# Autodesk Inventor assembly: WheelAssembly3.0
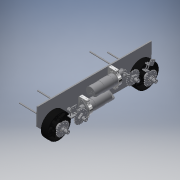
[picture p0: Inventor's stored thumbnail of the model, 180x180]
Saved by Autodesk Inventor 2017 (Build 210142000, 142)
## iProperties
Created: 2017-07-22
Part Number: WheelAssembly3.0
Document SubType Name: Assembly
Designer: User
Author: User
## Documents named in this file (17)
- C:\Robotics\CAD\2018-19_CAD\InvertedDriveTrain.iam
- C:\Robotics\CAD\COTSParts\Motors\Andymark 2964  NeveRest 40 Motor.ipt
- C:\Robotics\CAD\COTSParts\Tetrix\tetrix-motor-mounts-1.snapshot.1\Tetrex 2pc motor mount.ipt
- C:\Robotics\CAD\COTSParts\Actobotics\615 parts\615398.25inBoreBeveledGears.ipt
- C:\Robotics\CAD\2016-17_CAD\Custom COTS\4inax.ipt
- C:\Robotics\CAD\COTSParts\Actobotics\615 parts\615106Sprocket.5inBore.25inPitch24Teeth.ipt
- C:\Robotics\CAD\COTSParts\Actobotics\545 parts\545556SetScrewHub.77inPattern.ipt
- C:\Robotics\CAD\COTSParts\Wheels\4in Wheel Intergreated Hub 8mm Rev2.ipt
- C:\Robotics\CAD\COTSParts\Actobotics\Thrust Bearings\6655K13.ipt
- C:\Robotics\CAD\2018-19_CAD\InvertedDrivePlateOutside.ipt
- C:\Robotics\CAD\2018-19_CAD\InvertedDrivePlateInside.ipt
- C:\Robotics\CAD\2018-19_CAD\Offseason\WheelandSprocketComboHub2.ipt
- C:\Robotics\CAD\COTSParts\Actobotics\535 parts\535198Bearing.25ID.5OD.ipt
- C:\Robotics\CAD\2018-19_CAD\Offseason\Tensioner3.iam
- C:\Robotics\CAD\2018-19_CAD\Offseason\MotorFixedPositionMountInvertedDrive.ipt
- C:\Robotics\CAD\COTSParts\Actobotics\Collar.ipt
- C:\Robotics\CAD\COTSParts\Fasteners\6-32 SHCS x500.ipt
## Components (56 placed, 16 different names)
1. Andymark 2964  NeveRest 40 Motor:1 — Insert:3, Insert:6
2. Andymark 2964  NeveRest 40 Motor:2 — Insert:4, Insert:5
3. Tetrex 2pc motor mount:1 — Insert:3, Insert:79, Angle:8, Insert:84
4. Tetrex 2pc motor mount:2 — Insert:4, Insert:80, Angle:9, Insert:85
5. 615398.25inBoreBeveledGears:1 — Insert:5, Insert:44
6. 615398.25inBoreBeveledGears:2 — Insert:6, Insert:47
7. 615398.25inBoreBeveledGears:3 — Insert:77
8. 615398.25inBoreBeveledGears:4 — Insert:78
9. 4inax:1 — Insert:60, Mate:30
10. 4inax:2 — Insert:61
11. 615106Sprocket.5inBore.25inPitch24Teeth:2 — Insert:102, Insert:103, Insert:104
12. 4inax:3 — Insert:58, Mate:29
13. 4inax:4 — Insert:59
14. 545556SetScrewHub.77inPattern:4 — Insert:54
15. 4in Wheel Intergreated Hub 8mm Rev2:1 — Insert:65
16. 4in Wheel Intergreated Hub 8mm Rev2:2 — Insert:68
17. 545556SetScrewHub.77inPattern:7 — Insert:55
18. 615106Sprocket.5inBore.25inPitch24Teeth:3 — Insert:105, Insert:106, Insert:107
19. 6655K13:1 — Insert:64, Insert:78
20. 6655K13:2 — Insert:63, Insert:77
21. 6655K13:3 — Insert:44
22. 6655K13:4 — Insert:47
23. 615106Sprocket.5inBore.25inPitch24Teeth:4 — Insert:54, Mate:29
24. 615106Sprocket.5inBore.25inPitch24Teeth:5 — Insert:55, Mate:30
25. InvertedDrivePlateOutside:1 — Flush:1, Mate:24, Flush:2, Insert:58, Insert:59, Insert:60, Insert:61, Insert:71, Insert:72, Insert:73, Insert:74, Insert:75, Insert:76, Angle:10, Insert:81, Insert:82, Insert:83
26. InvertedDrivePlateInside:1 — Flush:1, Mate:24, Flush:2, Insert:63, Insert:64, Insert:79, Angle:8, Insert:80, Angle:9, Angle:11, Angle:12, Insert:90, Insert:91, Insert:92, Insert:93, Insert:98, Insert:99, Insert:100, Insert:101
27. WheelandSprocketComboHub2:1 — Insert:68, Insert:75, Insert:104, Mate:31
28. WheelandSprocketComboHub2:2 — Insert:65, Insert:76, Insert:107, Mate:32
29. 535198Bearing.25ID.5OD:1 — Insert:71, Insert:86
30. 535198Bearing.25ID.5OD:2 — Insert:74, Insert:89
31. 535198Bearing.25ID.5OD:3 — Insert:73, Insert:88
32. 535198Bearing.25ID.5OD:4 — Insert:72, Insert:87
33. Tensioner3:1 [sub-assembly] — Insert:82, Insert:83
34. Tensioner3:2 [sub-assembly] — Angle:10, Insert:81
35. MotorFixedPositionMountInvertedDrive:1 — Insert:84, Angle:11
36. MotorFixedPositionMountInvertedDrive:2 — Insert:85, Angle:12
37. Collar:1 — Insert:86
38. Collar:2 — Insert:87
39. Collar:3 — Insert:88
40. Collar:4 — Insert:89
41. Collar:5 — Insert:97
42. Collar:6 — Insert:96
43. Collar:7 — Insert:95
44. Collar:8 — Insert:94
45. 535198Bearing.25ID.5OD:5 — Insert:90, Insert:94
46. 535198Bearing.25ID.5OD:6 — Insert:91, Insert:95
47. 535198Bearing.25ID.5OD:7 — Insert:92, Insert:96
48. 535198Bearing.25ID.5OD:8 — Insert:93, Insert:97
49. 6-32 SHCS x500:1 — Insert:99
50. 6-32 SHCS x500:2 — Insert:98
51. 6-32 SHCS x500:3 — Insert:100
52. 6-32 SHCS x500:4 — Insert:101
53. 6-32 SHCS x500:5 — Insert:105, Mate:32
54. 6-32 SHCS x500:6 — Insert:106
55. 6-32 SHCS x500:7 — Insert:103
56. 6-32 SHCS x500:9 — Insert:102, Mate:31
## Relationships (65: Insert 53, Mate 5, Angle 5, Flush 2)
- Insert:3: Andymark 2964  NeveRest 40 Motor:1 ↔ Tetrex 2pc motor mount:1
- Insert:4: Andymark 2964  NeveRest 40 Motor:2 ↔ Tetrex 2pc motor mount:2
- Insert:5: Andymark 2964  NeveRest 40 Motor:2 ↔ 615398.25inBoreBeveledGears:1
- Insert:6: Andymark 2964  NeveRest 40 Motor:1 ↔ 615398.25inBoreBeveledGears:2
- Insert:44: 615398.25inBoreBeveledGears:1 ↔ 6655K13:3
- Insert:47: 615398.25inBoreBeveledGears:2 ↔ 6655K13:4
- Insert:54: 545556SetScrewHub.77inPattern:4 ↔ 615106Sprocket.5inBore.25inPitch24Teeth:4
- Insert:55: 545556SetScrewHub.77inPattern:7 ↔ 615106Sprocket.5inBore.25inPitch24Teeth:5
- Flush:1: InvertedDrivePlateOutside:1 ↔ InvertedDrivePlateInside:1
- Mate:24 (57.15 mm): InvertedDrivePlateOutside:1 ↔ InvertedDrivePlateInside:1
- Flush:2: InvertedDrivePlateOutside:1 ↔ InvertedDrivePlateInside:1
- Insert:58 (-6.35 mm): 4inax:3 ↔ InvertedDrivePlateOutside:1
- Insert:59 (-6.35 mm): 4inax:4 ↔ InvertedDrivePlateOutside:1
- Insert:60 (-6.35 mm): 4inax:1 ↔ InvertedDrivePlateOutside:1
- Insert:61 (-6.35 mm): 4inax:2 ↔ InvertedDrivePlateOutside:1
- Insert:63 (1.4224 mm): 6655K13:2 ↔ InvertedDrivePlateInside:1
- Insert:64 (-1.4224 mm): 6655K13:1 ↔ InvertedDrivePlateInside:1
- Insert:65: 4in Wheel Intergreated Hub 8mm Rev2:1 ↔ WheelandSprocketComboHub2:2
- Insert:68: 4in Wheel Intergreated Hub 8mm Rev2:2 ↔ WheelandSprocketComboHub2:1
- Insert:71: InvertedDrivePlateOutside:1 ↔ 535198Bearing.25ID.5OD:1
- Insert:72: InvertedDrivePlateOutside:1 ↔ 535198Bearing.25ID.5OD:4
- Insert:73: InvertedDrivePlateOutside:1 ↔ 535198Bearing.25ID.5OD:3
- Insert:74: InvertedDrivePlateOutside:1 ↔ 535198Bearing.25ID.5OD:2
- Insert:75 (1.27 mm): InvertedDrivePlateOutside:1 ↔ WheelandSprocketComboHub2:1
- Insert:76 (1.27 mm): InvertedDrivePlateOutside:1 ↔ WheelandSprocketComboHub2:2
- Insert:77: 615398.25inBoreBeveledGears:3 ↔ 6655K13:2
- Mate:29: 4inax:3 ↔ 615106Sprocket.5inBore.25inPitch24Teeth:4
- Insert:78: 615398.25inBoreBeveledGears:4 ↔ 6655K13:1
- Mate:30: 4inax:1 ↔ 615106Sprocket.5inBore.25inPitch24Teeth:5
- Insert:79: Tetrex 2pc motor mount:1 ↔ InvertedDrivePlateInside:1
- Angle:8 (0 deg): Tetrex 2pc motor mount:1 ↔ InvertedDrivePlateInside:1
- Insert:80: Tetrex 2pc motor mount:2 ↔ InvertedDrivePlateInside:1
- Angle:9 (0 deg): Tetrex 2pc motor mount:2 ↔ InvertedDrivePlateInside:1
- Angle:10 (-62 deg): InvertedDrivePlateOutside:1 ↔ Tensioner3:2
- Insert:81: InvertedDrivePlateOutside:1 ↔ Tensioner3:2
- Insert:82: InvertedDrivePlateOutside:1 ↔ Tensioner3:1
- Insert:83: InvertedDrivePlateOutside:1 ↔ Tensioner3:1
- Insert:84: Tetrex 2pc motor mount:1 ↔ MotorFixedPositionMountInvertedDrive:1
- Angle:11 (180 deg): InvertedDrivePlateInside:1 ↔ MotorFixedPositionMountInvertedDrive:1
- Insert:85: Tetrex 2pc motor mount:2 ↔ MotorFixedPositionMountInvertedDrive:2
- Angle:12 (180 deg): InvertedDrivePlateInside:1 ↔ MotorFixedPositionMountInvertedDrive:2
- Insert:86: 535198Bearing.25ID.5OD:1 ↔ Collar:1
- Insert:87: 535198Bearing.25ID.5OD:4 ↔ Collar:2
- Insert:88: 535198Bearing.25ID.5OD:3 ↔ Collar:3
- Insert:89: 535198Bearing.25ID.5OD:2 ↔ Collar:4
- Insert:90: InvertedDrivePlateInside:1 ↔ 535198Bearing.25ID.5OD:5
- Insert:91: InvertedDrivePlateInside:1 ↔ 535198Bearing.25ID.5OD:6
- Insert:92: InvertedDrivePlateInside:1 ↔ 535198Bearing.25ID.5OD:7
- Insert:93: InvertedDrivePlateInside:1 ↔ 535198Bearing.25ID.5OD:8
- Insert:94: Collar:8 ↔ 535198Bearing.25ID.5OD:5
- Insert:95: Collar:7 ↔ 535198Bearing.25ID.5OD:6
- Insert:96: Collar:6 ↔ 535198Bearing.25ID.5OD:7
- Insert:97: Collar:5 ↔ 535198Bearing.25ID.5OD:8
- Insert:98: InvertedDrivePlateInside:1 ↔ 6-32 SHCS x500:2
- Insert:99: InvertedDrivePlateInside:1 ↔ 6-32 SHCS x500:1
- Insert:100: InvertedDrivePlateInside:1 ↔ 6-32 SHCS x500:3
- Insert:101: InvertedDrivePlateInside:1 ↔ 6-32 SHCS x500:4
- Insert:102: 615106Sprocket.5inBore.25inPitch24Teeth:2 ↔ 6-32 SHCS x500:9
- Insert:103: 615106Sprocket.5inBore.25inPitch24Teeth:2 ↔ 6-32 SHCS x500:7
- Insert:104: 615106Sprocket.5inBore.25inPitch24Teeth:2 ↔ WheelandSprocketComboHub2:1
- Mate:31: WheelandSprocketComboHub2:1 ↔ 6-32 SHCS x500:9
- Insert:105: 615106Sprocket.5inBore.25inPitch24Teeth:3 ↔ 6-32 SHCS x500:5
- Insert:106: 615106Sprocket.5inBore.25inPitch24Teeth:3 ↔ 6-32 SHCS x500:6
- Insert:107: 615106Sprocket.5inBore.25inPitch24Teeth:3 ↔ WheelandSprocketComboHub2:2
- Mate:32: WheelandSprocketComboHub2:2 ↔ 6-32 SHCS x500:5
